# Autodesk Inventor assembly: Foerderband_V1
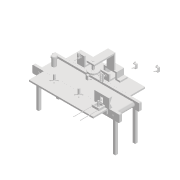
[picture p0: Inventor's stored thumbnail of the model, 180x180]
Saved by Autodesk Inventor 2020 (Build 240168000, 168)
## iProperties
Created: 2020-03-15
Part Number: Foerderband_V1
Document SubType Name: Assembly
Designer: franz
Author: franz
## Documents named in this file (8)
- E:\Privat\Projekte\SPS_Training\Unity_SPS_Simulation\Unity_SPS_Schrittkette\CAD\Foerderband_V1\Foerderband_V1.iam
- E:\Privat\Projekte\SPS_Training\Unity_SPS_Simulation\Unity_SPS_Schrittkette\CAD\Foerderband_V1\Foerderband_150cm\Foerderband_150cm.iam
- E:\Privat\Projekte\SPS_Training\Unity_SPS_Simulation\Unity_SPS_Schrittkette\CAD\Foerderband_V1\Lackieranlage\Lackieranlage.iam
- E:\Privat\Projekte\SPS_Training\Unity_SPS_Simulation\Unity_SPS_Schrittkette\CAD\Foerderband_V1\Drehgreifer\Drehgreifer.iam
- E:\Privat\Projekte\SPS_Training\Unity_SPS_Simulation\Unity_SPS_Schrittkette\CAD\Foerderband_V1\Scanner\Scanner.iam
- E:\Privat\Projekte\SPS_Training\Unity_SPS_Simulation\Unity_SPS_Schrittkette\CAD\Foerderband_V1\Sortierer\Sortierer.iam
- E:\Privat\Projekte\SPS_Training\Unity_SPS_Simulation\Unity_SPS_Schrittkette\CAD\Foerderband_V1\Positionssensor\Positionssensor.iam
- E:\Privat\Projekte\SPS_Training\Unity_SPS_Simulation\Unity_SPS_Schrittkette\CAD\Foerderband_V1\Objekt\Objekt.iam
## Components (9 placed, 7 different names)
1. Foerderband_150cm:1 [sub-assembly] — Passend:1, Fluchtend:1, Passend:2, Passend:3, Passend:4, Fluchtend:2, Passend:5, Passend:6, Fluchtend:3, Passend:7, Passend:8, Passend:9, Passend:10, Passend:11, Passend:12, Fluchtend:6, Passend:13, Passend:15
2. Lackieranlage:1 [sub-assembly] — Passend:1, Fluchtend:1, Passend:2, Fluchtend:4
3. Drehgreifer:1 [sub-assembly] — Passend:5, Passend:6, Fluchtend:3
4. Scanner:1 [sub-assembly] — Passend:3, Passend:4, Fluchtend:2, Fluchtend:5
5. Sortierer:1 [sub-assembly] — Passend:13, Passend:14, Passend:15
6. Positionssensor:1 [sub-assembly] — Passend:7, Passend:10, Fluchtend:4
7. Positionssensor:2 [sub-assembly] — Passend:8, Passend:11, Fluchtend:5
8. Positionssensor:3 [sub-assembly] — Passend:9, Passend:12, Fluchtend:6, Passend:14
9. Objekt:1 [sub-assembly]
## Relationships (21: Mate 15, Flush 6)
- Passend:1 [Mate]: Foerderband_150cm:1 ↔ Lackieranlage:1
- Fluchtend:1 [Flush] (200 mm): Foerderband_150cm:1 ↔ Lackieranlage:1
- Passend:2 [Mate] (20 mm): Foerderband_150cm:1 ↔ Lackieranlage:1
- Passend:3 [Mate]: Foerderband_150cm:1 ↔ Scanner:1
- Passend:4 [Mate] (20 mm): Foerderband_150cm:1 ↔ Scanner:1
- Fluchtend:2 [Flush] (700 mm): Foerderband_150cm:1 ↔ Scanner:1
- Passend:5 [Mate]: Foerderband_150cm:1 ↔ Drehgreifer:1
- Passend:6 [Mate] (120 mm): Foerderband_150cm:1 ↔ Drehgreifer:1
- Fluchtend:3 [Flush] (575 mm): Foerderband_150cm:1 ↔ Drehgreifer:1
- Passend:7 [Mate]: Foerderband_150cm:1 ↔ Positionssensor:1
- Passend:8 [Mate]: Foerderband_150cm:1 ↔ Positionssensor:2
- Passend:9 [Mate]: Foerderband_150cm:1 ↔ Positionssensor:3
- Passend:10 [Mate] (50 mm): Foerderband_150cm:1 ↔ Positionssensor:1
- Passend:11 [Mate] (50 mm): Foerderband_150cm:1 ↔ Positionssensor:2
- Passend:12 [Mate] (65 mm): Foerderband_150cm:1 ↔ Positionssensor:3
- Fluchtend:4 [Flush] (60 mm): Lackieranlage:1 ↔ Positionssensor:1
- Fluchtend:5 [Flush] (60 mm): Scanner:1 ↔ Positionssensor:2
- Fluchtend:6 [Flush] (100 mm): Foerderband_150cm:1 ↔ Positionssensor:3
- Passend:13 [Mate]: Foerderband_150cm:1 ↔ Sortierer:1
- Passend:14 [Mate] (35 mm): Sortierer:1 ↔ Positionssensor:3
- Passend:15 [Mate] (20 mm): Foerderband_150cm:1 ↔ Sortierer:1
